# Autodesk Inventor assembly: okragla duza
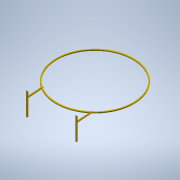
[picture p0: Inventor's stored thumbnail of the model, 180x180]
Saved by Autodesk Inventor 2021 (Build 250183000, 183)
## iProperties
Created: 2024-04-18
Part Number: okragla duza
Document SubType Name: Assembly
Designer: Michal
Author: Michal
## Documents named in this file (6)
- C:\Users\Michal\Documents\GitHub\PNW_PhotoBoothFrame_3D\okragla duza.iam
- C:\Users\Michal\Documents\GitHub\PNW_PhotoBoothFrame_3D\Stopa v4.iam
- C:\Users\Michal\Documents\GitHub\PNW_PhotoBoothFrame_3D\Luk R2000.ipt
- C:\Users\Michal\Documents\GitHub\PNW_PhotoBoothFrame_3D\Lacznik zaokraglony sruby.iam
- C:\Users\Michal\Documents\GitHub\PNW_PhotoBoothFrame_3D\noga do okraglej duzej L.ipt
- C:\Users\Michal\Documents\GitHub\PNW_PhotoBoothFrame_3D\noga do okraglej duzej P.ipt
## Components (8 placed, 5 different names)
1. Luk R2000:1 — Flush:19, Mate:20, Mate:21, Mate:27, Mate:28, Flush:26, Flush:27, Mate:35
2. Lacznik zaokraglony sruby:1 [sub-assembly] — Flush:19, Mate:20, Mate:21, Flush:21
3. Luk R2000:2 — Mate:24, Mate:26, Mate:29, Mate:30
4. Lacznik zaokraglony sruby:2 [sub-assembly] — Mate:24, Mate:26, Flush:21, Mate:27, Mate:28, Flush:22
5. noga do okraglej duzej L:1 — Flush:23, Mate:30, Mate:31, Flush:24, Mate:32
6. noga do okraglej duzej P:1 — Flush:22, Mate:29, Flush:23, Mate:33, Flush:25, Mate:34
7. Stopa v4:3 [sub-assembly] — Mate:31, Flush:24, Mate:32
8. Stopa v4:4 [sub-assembly] — Mate:33, Flush:25, Mate:34
## Relationships (22: Mate 13, Flush 9)
- Flush:19: Luk R2000:1 ↔ Lacznik zaokraglony sruby:1
- Mate:20: Luk R2000:1 ↔ Lacznik zaokraglony sruby:1
- Mate:21: Luk R2000:1 ↔ Lacznik zaokraglony sruby:1
- [Flush]: Luk R2000:2 ↔ Lacznik zaokraglony sruby:2
- Mate:24: Luk R2000:2 ↔ Lacznik zaokraglony sruby:2
- Mate:26: Luk R2000:2 ↔ Lacznik zaokraglony sruby:2
- Flush:21: Lacznik zaokraglony sruby:1 ↔ Lacznik zaokraglony sruby:2
- Mate:27: Luk R2000:1 ↔ Lacznik zaokraglony sruby:2
- Mate:28: Luk R2000:1 ↔ Lacznik zaokraglony sruby:2
- Flush:22: Lacznik zaokraglony sruby:2 ↔ noga do okraglej duzej P:1
- Mate:29: Luk R2000:2 ↔ noga do okraglej duzej P:1
- Flush:23: noga do okraglej duzej L:1 ↔ noga do okraglej duzej P:1
- Mate:30: Luk R2000:2 ↔ noga do okraglej duzej L:1
- Mate:31: noga do okraglej duzej L:1 ↔ Stopa v4:3
- Flush:24: noga do okraglej duzej L:1 ↔ Stopa v4:3
- Mate:32: noga do okraglej duzej L:1 ↔ Stopa v4:3
- Mate:33: noga do okraglej duzej P:1 ↔ Stopa v4:4
- Flush:25: noga do okraglej duzej P:1 ↔ Stopa v4:4
- Mate:34: noga do okraglej duzej P:1 ↔ Stopa v4:4
- Flush:26: Luk R2000:1
- Flush:27: Luk R2000:1
- Mate:35: Luk R2000:1
## Named parameters: d125_d120 = 0 mm
